# Autodesk Inventor assembly: cino_build_aluminum
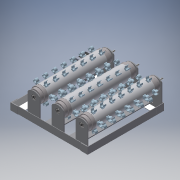
[picture p0: Inventor's stored thumbnail of the model, 180x180]
Saved by Autodesk Inventor 2018 (Build 220112000, 112)
## iProperties
Created: 2018-10-27
Part Number: cino_build_aluminum
Document SubType Name: Assembly
Designer: Fredy Espana C
Author: Fredy Espana C
## Documents named in this file (18)
- C:\Users\My User\Documents\Trabajos UVG\8vo. Semestre\Diseño Mecánico 2\Proyecto\Inventor Files\Clino\cino_build_aluminum.iam
- C:\Users\My User\Documents\Trabajos UVG\8vo. Semestre\Diseño Mecánico 2\Proyecto\Inventor Files\Clino\Lframe_280mm.ipt
- C:\Users\My User\Documents\Trabajos UVG\8vo. Semestre\Diseño Mecánico 2\Proyecto\Inventor Files\Clino\Lframe_350mm.ipt
- C:\Users\My User\Documents\Trabajos UVG\8vo. Semestre\Diseño Mecánico 2\Proyecto\Inventor Files\Clino\Lframe_corner.ipt
- C:\Users\My User\Documents\Trabajos UVG\8vo. Semestre\Diseño Mecánico 2\Proyecto\Inventor Files\Clino\platen_286mm.ipt
- C:\Users\My User\Documents\Trabajos UVG\8vo. Semestre\Diseño Mecánico 2\Proyecto\Inventor Files\Clino\platen_support.ipt
- C:\Users\My User\Documents\Trabajos UVG\8vo. Semestre\Diseño Mecánico 2\Proyecto\Inventor Files\Clino\nema17.ipt
- C:\Users\My User\Documents\Trabajos UVG\8vo. Semestre\Diseño Mecánico 2\Proyecto\Inventor Files\Clino\2inpvc_pipe.ipt
- C:\Users\My User\Documents\Trabajos UVG\8vo. Semestre\Diseño Mecánico 2\Proyecto\Inventor Files\Clino\pipe_holder.ipt
- C:\Users\My User\Documents\Trabajos UVG\8vo. Semestre\Diseño Mecánico 2\Proyecto\Inventor Files\Clino\motor_bases.ipt
- C:\Users\My User\Documents\Trabajos UVG\8vo. Semestre\Diseño Mecánico 2\Proyecto\Inventor Files\Clino\snap_grip.ipt
- C:\Users\My User\Documents\Trabajos UVG\8vo. Semestre\Diseño Mecánico 2\Proyecto\Inventor Files\Clino\cino_build_aluminum\Design Accelerator\Bearing1.iam
- C:\Users\My User\Documents\Trabajos UVG\8vo. Semestre\Diseño Mecánico 2\Proyecto\Inventor Files\Clino\cino_build_aluminum\Design Accelerator\Bearing2.iam
- C:\Users\My User\Documents\Trabajos UVG\8vo. Semestre\Diseño Mecánico 2\Proyecto\Inventor Files\Clino\cino_build_aluminum\Design Accelerator\Bearing3.iam
- C:\Users\My User\Documents\Trabajos UVG\8vo. Semestre\Diseño Mecánico 2\Proyecto\Inventor Files\Clino\cino_build_aluminum\Design Accelerator\Bearing4.iam
- C:\Users\My User\Documents\Trabajos UVG\8vo. Semestre\Diseño Mecánico 2\Proyecto\Inventor Files\Clino\cino_build_aluminum\Design Accelerator\Bearing5.iam
- C:\Users\My User\Documents\Trabajos UVG\8vo. Semestre\Diseño Mecánico 2\Proyecto\Inventor Files\Clino\cino_build_aluminum\Design Accelerator\Bearing6.iam
- C:\Users\My User\Documents\Trabajos UVG\8vo. Semestre\Diseño Mecánico 2\Proyecto\Inventor Files\Clino\shaft.ipt
## Components (144 placed, 12 different names)
1. Lframe_280mm:1 — Mate:1, Mate:2, Flush:1, Mate:3, Mate:4, Flush:2, Mate:9, Mate:12, Mate:41, Mate:44, Mate:46, Mate:53, Mate:55
2. Lframe_350mm:1 — Mate:1, Mate:2, Flush:1, Flush:3, Mate:6, Mate:8, Flush:4, Mate:10, Flush:5, Mate:18, Mate:19, Mate:25, Mate:26, Mate:27, Mate:28, Mate:30, Mate:31, Mate:35
3. Lframe_350mm:2 — Mate:3, Mate:4, Flush:2, Mate:5, Mate:11, Flush:6, Mate:14, Flush:7, Mate:16, Mate:17, Mate:21, Mate:22, Mate:23, Mate:24, Mate:34, Mate:41, Mate:42, Mate:43, Mate:47, Mate:52, Mate:56
4. Lframe_280mm:2 — Mate:5, Flush:3, Mate:6, Mate:7, Mate:13, Mate:15, Mate:20
5. Lframe_corner:1 — Mate:11, Mate:12, Flush:6
6. Lframe_corner:2 — Mate:13, Mate:14, Flush:7
7. Lframe_corner:3 — Mate:7, Mate:8, Flush:4
8. Lframe_corner:4 — Mate:9, Mate:10, Flush:5
9. platen_support:1 — Mate:23, Mate:24, Mate:38, Mate:61, Mate:62, Mate:74
10. platen_support:2 — Mate:21, Mate:22, Mate:33, Mate:59, Mate:60, Mate:72
11. platen_support:3 — Mate:15, Mate:16, Mate:17, Mate:58, Flush:11
12. platen_support:4 — Mate:26, Mate:28, Mate:37, Mate:63, Mate:64
13. platen_support:5 — Mate:25, Mate:27, Mate:32, Mate:36, Mate:65, Mate:66
14. platen_support:6 — Mate:18, Mate:19, Mate:20, Mate:29, Mate:67, Mate:68, Mate:69
15. platen_286mm:1 — Mate:29, Mate:30, Mate:31, Mate:32, Mate:33
16. platen_286mm:2 — Mate:34, Mate:35, Mate:36, Mate:37, Mate:38
17. nema17:1 — Mate:54, Mate:55, Mate:56
18. 2inpvc_pipe:2 — Insert:5, Insert:6, Insert:7, Mate:57, Mate:70
19. pipe_holder:3 — Insert:5, Flush:10
20. pipe_holder:4 — Insert:6, Insert:7, Cylindrical:2, Mate:69
21. motor_bases:1 — Mate:42, Mate:43, Mate:44, Mate:45
22. motor_bases:2 — Mate:45, Mate:46, Mate:47, Mate:51
23. motor_bases:3 — Mate:50, Flush:8, Flush:9, Mate:52, Mate:53, Mate:54
24. motor_bases:4 — Mate:50, Flush:8, Flush:9, Mate:51
25. Bearing:1 [sub-assembly] — Mate:58, Flush:11, Cylindrical:1
26. Bearing:2 [sub-assembly] — Mate:59, Mate:60, Cylindrical:3
27. Bearing:3 [sub-assembly] — Mate:61, Mate:62
28. Bearing:4 [sub-assembly] — Mate:63, Mate:64, Cylindrical:4, Flush:15
29. Bearing:5 [sub-assembly] — Mate:65, Mate:66, Flush:14
30. Bearing:6 [sub-assembly] — Mate:67, Mate:68, Flush:12, Flush:13
31. shaft:1 — Cylindrical:1, Flush:12, Flush:13, Cylindrical:2
32. shaft:2 — Cylindrical:4, Flush:15, Cylindrical:6
33. shaft:3 — Cylindrical:3, Flush:14, Cylindrical:5
34. 2inpvc_pipe:3 — Insert:8, Insert:9, Mate:71
35. 2inpvc_pipe:4 — Insert:10, Insert:11, Mate:73
36. pipe_holder:5 — Insert:8, Flush:16, Cylindrical:5, Mate:72
37. pipe_holder:6 — Insert:10, Flush:17, Cylindrical:6, Mate:74
38. pipe_holder:7 — Insert:9
39. pipe_holder:8 — Insert:11
40. snap_grip:1 — Flush:10, Mate:57
41. snap_grip:2
42. snap_grip:3
43. snap_grip:4
44. snap_grip:5 — Mate:70
45. snap_grip:6
46. snap_grip:7
47. snap_grip:8
48. snap_grip:9
49. snap_grip:10
50. snap_grip:11
51. snap_grip:12
52. snap_grip:13
53. snap_grip:14
54. snap_grip:15
55. snap_grip:16
56. snap_grip:17
57. snap_grip:18
58. snap_grip:19
59. snap_grip:20
60. snap_grip:21
61. snap_grip:22
62. snap_grip:23
63. snap_grip:24
64. snap_grip:25
65. snap_grip:26
66. snap_grip:27
67. snap_grip:28
68. snap_grip:29
69. snap_grip:30
70. snap_grip:31
71. snap_grip:32
72. snap_grip:33
73. snap_grip:34
74. snap_grip:35
75. snap_grip:36 — Mate:71, Flush:16
76. snap_grip:38
77. snap_grip:39
78. snap_grip:40
79. snap_grip:41
80. snap_grip:42
81. snap_grip:43
82. snap_grip:44
83. snap_grip:45
84. snap_grip:46
85. snap_grip:47
86. snap_grip:48
87. snap_grip:49
88. snap_grip:50
89. snap_grip:51
90. snap_grip:52
91. snap_grip:53
92. snap_grip:54
93. snap_grip:55
94. snap_grip:56
95. snap_grip:57
96. snap_grip:58
97. snap_grip:59
98. snap_grip:60
99. snap_grip:61
100. snap_grip:62
101. snap_grip:63
102. snap_grip:64
103. snap_grip:65
104. snap_grip:66
105. snap_grip:67
106. snap_grip:68
107. snap_grip:69
108. snap_grip:70
109. snap_grip:71
110. snap_grip:37 — Mate:73, Flush:17
111. snap_grip:72
112. snap_grip:73
113. snap_grip:74
114. snap_grip:75
115. snap_grip:76
116. snap_grip:77
117. snap_grip:78
118. snap_grip:79
119. snap_grip:80
120. snap_grip:81
121. snap_grip:82
122. snap_grip:83
123. snap_grip:84
124. snap_grip:85
125. snap_grip:86
126. snap_grip:87
127. snap_grip:88
128. snap_grip:89
129. snap_grip:90
130. snap_grip:91
131. snap_grip:92
132. snap_grip:93
133. snap_grip:94
134. snap_grip:95
135. snap_grip:96
136. snap_grip:97
137. snap_grip:98
138. snap_grip:99
139. snap_grip:100
140. snap_grip:101
141. snap_grip:102
142. snap_grip:103
143. snap_grip:104
144. snap_grip:105
## Component patterns: (7 elements), (7 elements), (7 elements), (5 elements, first: snap_grip:1), Component Pattern 3:2 (5 elements), Component Pattern 3:3 (5 elements), Component Pattern 3:4 (5 elements), Component Pattern 3:5 (5 elements), Component Pattern 3:6 (5 elements), Component Pattern 3:7 (5 elements), (5 elements, first: snap_grip:36), Component Pattern 5:2 (5 elements), Component Pattern 5:3 (5 elements), Component Pattern 5:4 (5 elements), Component Pattern 5:5 (5 elements), Component Pattern 5:6 (5 elements), Component Pattern 5:7 (5 elements), (5 elements, first: snap_grip:37), Component Pattern 7:2 (5 elements), Component Pattern 7:3 (5 elements), Component Pattern 7:4 (5 elements), Component Pattern 7:5 (5 elements), Component Pattern 7:6 (5 elements), Component Pattern 7:7 (5 elements)
## Relationships (100: Mate 70, Flush 17, Insert 7, CylindricalJoint 6)
- Mate:1: Lframe_280mm:1 ↔ Lframe_350mm:1
- Mate:2: Lframe_280mm:1 ↔ Lframe_350mm:1
- Flush:1: Lframe_280mm:1 ↔ Lframe_350mm:1
- Mate:3: Lframe_280mm:1 ↔ Lframe_350mm:2
- Mate:4: Lframe_280mm:1 ↔ Lframe_350mm:2
- Flush:2: Lframe_280mm:1 ↔ Lframe_350mm:2
- Mate:5: Lframe_350mm:2 ↔ Lframe_280mm:2
- Flush:3: Lframe_350mm:1 ↔ Lframe_280mm:2
- Mate:6: Lframe_350mm:1 ↔ Lframe_280mm:2
- Mate:7: Lframe_280mm:2 ↔ Lframe_corner:3
- Mate:8: Lframe_350mm:1 ↔ Lframe_corner:3
- Flush:4: Lframe_350mm:1 ↔ Lframe_corner:3
- Mate:9: Lframe_280mm:1 ↔ Lframe_corner:4
- Mate:10: Lframe_350mm:1 ↔ Lframe_corner:4
- Flush:5: Lframe_350mm:1 ↔ Lframe_corner:4
- Mate:11: Lframe_350mm:2 ↔ Lframe_corner:1
- Mate:12: Lframe_280mm:1 ↔ Lframe_corner:1
- Flush:6: Lframe_350mm:2 ↔ Lframe_corner:1
- Mate:13: Lframe_280mm:2 ↔ Lframe_corner:2
- Mate:14: Lframe_350mm:2 ↔ Lframe_corner:2
- Flush:7: Lframe_350mm:2 ↔ Lframe_corner:2
- Mate:15: Lframe_280mm:2 ↔ platen_support:3
- Mate:16: Lframe_350mm:2 ↔ platen_support:3
- Mate:17: Lframe_350mm:2 ↔ platen_support:3
- Mate:18: Lframe_350mm:1 ↔ platen_support:6
- Mate:19: Lframe_350mm:1 ↔ platen_support:6
- Mate:20: Lframe_280mm:2 ↔ platen_support:6
- Mate:21: Lframe_350mm:2 ↔ platen_support:2
- Mate:22: Lframe_350mm:2 ↔ platen_support:2
- Mate:23: Lframe_350mm:2 ↔ platen_support:1
- Mate:24: Lframe_350mm:2 ↔ platen_support:1
- Mate:25: Lframe_350mm:1 ↔ platen_support:5
- Mate:26: Lframe_350mm:1 ↔ platen_support:4
- Mate:27: Lframe_350mm:1 ↔ platen_support:5
- Mate:28: Lframe_350mm:1 ↔ platen_support:4
- Mate:29: platen_support:6 ↔ platen_286mm:1
- Mate:30: Lframe_350mm:1 ↔ platen_286mm:1
- Mate:31: Lframe_350mm:1 ↔ platen_286mm:1
- Mate:32: platen_support:5 ↔ platen_286mm:1
- Mate:33: platen_support:2 ↔ platen_286mm:1
- Mate:34: Lframe_350mm:2 ↔ platen_286mm:2
- Mate:35: Lframe_350mm:1 ↔ platen_286mm:2
- Mate:36: platen_support:5 ↔ platen_286mm:2
- Mate:37: platen_support:4 ↔ platen_286mm:2
- Mate:38: platen_support:1 ↔ platen_286mm:2
- Insert:5: 2inpvc_pipe:2 ↔ pipe_holder:3
- Insert:6: 2inpvc_pipe:2 ↔ pipe_holder:4
- Mate:41: Lframe_280mm:1 ↔ Lframe_350mm:2
- Mate:42: Lframe_350mm:2 ↔ motor_bases:1
- Mate:43: Lframe_350mm:2 ↔ motor_bases:1
- Mate:44: Lframe_280mm:1 ↔ motor_bases:1
- Mate:45: motor_bases:1 ↔ motor_bases:2
- Mate:46: Lframe_280mm:1 ↔ motor_bases:2
- Mate:47: Lframe_350mm:2 ↔ motor_bases:2
- Mate:50: motor_bases:3 ↔ motor_bases:4
- Flush:8: motor_bases:3 ↔ motor_bases:4
- Flush:9: motor_bases:3 ↔ motor_bases:4
- Mate:51: motor_bases:2 ↔ motor_bases:4
- Mate:52: Lframe_350mm:2 ↔ motor_bases:3
- Mate:53: Lframe_280mm:1 ↔ motor_bases:3
- Mate:54: nema17:1 ↔ motor_bases:3
- Mate:55: Lframe_280mm:1 ↔ nema17:1
- Mate:56: Lframe_350mm:2 ↔ nema17:1
- Insert:7: 2inpvc_pipe:2 ↔ pipe_holder:4
- Flush:10 (25 mm): pipe_holder:3 ↔ snap_grip:1
- Mate:57: 2inpvc_pipe:2 ↔ snap_grip:1
- Mate:58: platen_support:3 ↔ Bearing:1
- Flush:11 (6 mm): platen_support:3 ↔ Bearing:1
- Mate:59: platen_support:2 ↔ Bearing:2
- Mate:60: platen_support:2 ↔ Bearing:2
- Mate:61: platen_support:1 ↔ Bearing:3
- Mate:62: platen_support:1 ↔ Bearing:3
- Mate:63: platen_support:4 ↔ Bearing:4
- Mate:64: platen_support:4 ↔ Bearing:4
- Mate:65: platen_support:5 ↔ Bearing:5
- Mate:66: platen_support:5 ↔ Bearing:5
- Mate:67: platen_support:6 ↔ Bearing:6
- Mate:68: platen_support:6 ↔ Bearing:6
- Cylindrical:1: Bearing:1 ↔ shaft:1
- Flush:12: Bearing:6 ↔ shaft:1
- Flush:13: Bearing:6 ↔ shaft:1
- Cylindrical:2: pipe_holder:4 ↔ shaft:1
- Mate:69 (3 mm): platen_support:6 ↔ pipe_holder:4
- Cylindrical:3: Bearing:2 ↔ shaft:3
- Flush:14: Bearing:5 ↔ shaft:3
- Cylindrical:4: Bearing:4 ↔ shaft:2
- Flush:15: Bearing:4 ↔ shaft:2
- Mate:70: 2inpvc_pipe:2 ↔ snap_grip:5
- Insert:8: 2inpvc_pipe:3 ↔ pipe_holder:5
- Insert:9: 2inpvc_pipe:3 ↔ pipe_holder:7
- Insert:10: 2inpvc_pipe:4 ↔ pipe_holder:6
- Insert:11: 2inpvc_pipe:4 ↔ pipe_holder:8
- Mate:71: 2inpvc_pipe:3 ↔ snap_grip:36
- Flush:16 (25 mm): pipe_holder:5 ↔ snap_grip:36
- Cylindrical:5: shaft:3 ↔ pipe_holder:5
- Mate:72 (3.5 mm): platen_support:2 ↔ pipe_holder:5
- Mate:73: 2inpvc_pipe:4 ↔ snap_grip:37
- Flush:17 (25 mm): pipe_holder:6 ↔ snap_grip:37
- Cylindrical:6: shaft:2 ↔ pipe_holder:6
- Mate:74 (3.5 mm): platen_support:1 ↔ pipe_holder:6
